# Autodesk Inventor assembly: Bloc roue
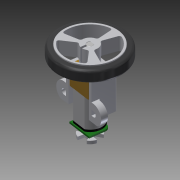
[picture p0: Inventor's stored thumbnail of the model, 180x180]
Saved by Autodesk Inventor 2014 SP2 (Build 180246200, 246)
## iProperties
Created: 2015-03-17
Part Number: Bloc roue
Document SubType Name: Assembly
Designer: sd
Mass: 25.2343 g
Surface Area: 66.5863 cm^2
Volume: 6.66012 cm^3
Density: 3.78886 g/cm^3
Author: sd
## Documents named in this file (5)
- D:\Utilisateurs\sd\Mes documents\SVN\projets-gei\Dumber 2015\Mecanique\Bloc roue.iam
- D:\Utilisateurs\sd\Mes documents\SVN\projets-gei\Dumber 2015\Mecanique\moteur.iam
- D:\Utilisateurs\sd\Mes documents\SVN\projets-gei\Dumber 2015\Mecanique\roue.iam
- D:\Utilisateurs\sd\Mes documents\SVN\projets-gei\Dumber 2015\Mecanique\helice encodeur.ipt
- D:\Utilisateurs\sd\Mes documents\SVN\projets-gei\Dumber 2015\Mecanique\Platine encodeur.ipt
## Components (4 placed, 4 different names)
1. moteur:1 [sub-assembly] — Placage:1, Angle:1, Affleurement:1, Placage:2, Affleurement:2, Placage:3, Affleurement:3, Placage:4
2. roue:1 [sub-assembly] — Placage:1, Angle:1, Affleurement:1
3. helice encodeur:1 — Affleurement:3, Placage:4
4. Platine encodeur:1 — Placage:2, Affleurement:2, Placage:3
## Relationships (8: Mate 4, Flush 3, Angle 1)
- Placage:1 [Mate]: moteur:1 ↔ roue:1
- Angle:1 (0 deg): moteur:1 ↔ roue:1
- Affleurement:1 [Flush]: moteur:1 ↔ roue:1
- Placage:2 [Mate]: moteur:1 ↔ Platine encodeur:1
- Affleurement:2 [Flush] (0.3 mm): moteur:1 ↔ Platine encodeur:1
- Placage:3 [Mate] (0.25 mm): moteur:1 ↔ Platine encodeur:1
- Affleurement:3 [Flush]: moteur:1 ↔ helice encodeur:1
- Placage:4 [Mate]: moteur:1 ↔ helice encodeur:1
